# Autodesk Inventor assembly: Assembly1
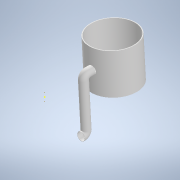
[picture p0: Inventor's stored thumbnail of the model, 180x180]
Saved by Autodesk Inventor 2021 (Build 250183000, 183)
## iProperties
Created: 2021-07-06
Part Number: Assembly1
Document SubType Name: Assembly
Designer: Nishat
Author: Nishat
## Documents named in this file (3)
- D:\exploration\virtual\virtual\Assembly1.iam
- D:\exploration\virtual\virtual\Part1.ipt
- D:\exploration\virtual\virtual\pipe.ipt
## Components (2 placed, 2 different names)
1. pipe:1 — Mate:1, Rigid:2
2. Part1:2 — Mate:1, Rigid:2
## Relationships (2: Mate 1, WeldJoint 1)
- Mate:1: pipe:1 ↔ Part1:2
- Rigid:2 [WeldJoint]: pipe:1 ↔ Part1:2
